# Autodesk Inventor assembly: POM_T5_03
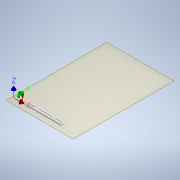
[picture p0: Inventor's stored thumbnail of the model, 180x180]
Saved by Autodesk Inventor 2020 (Build 240168000, 168)
## iProperties
Created: 2021-08-27
Part Number: POM_T5_03
Document SubType Name: Assembly
Designer: Masato
Author: Masato
## Documents named in this file (6)
- C:\Inventor\OpenPlatform_ver3_0\cam\POM_T5_03.iam
- C:\Inventor\OpenPlatform_ver3_0\cam\Disposable_Board.ipt
- C:\Inventor\OpenPlatform_ver3_0\JIG\BackLink_diagonal_jig.ipt
- C:\Inventor\OpenPlatform_ver3_0\JIG\FrontLink_diagonal_jig.ipt
- C:\Inventor\OpenPlatform_ver3_0\JIG\Foot_root_block_JIG.ipt
- C:\Inventor\OpenPlatform_ver3_0\JIG\Leg_joint_yaw_frame_JIG.ipt
## Components (5 placed, 5 different names)
1. Disposable_Board:1 — メイト:2, メイト:1, フラッシュ:1, フラッシュ:2, メイト:7, フラッシュ:6, メイト:17, フラッシュ:7, メイト:22, フラッシュ:8, メイト:27, フラッシュ:9, フラッシュ:10
2. FrontLink_diagonal_jig:1 — メイト:7, フラッシュ:6, メイト:18, メイト:28
3. BackLink_diagonal_jig:2 — メイト:17, フラッシュ:7, メイト:18
4. Foot_root_block_JIG:1 — メイト:22, フラッシュ:8, メイト:28, メイト:29
5. Leg_joint_yaw_frame_JIG:1 — メイト:27, フラッシュ:9, フラッシュ:10, メイト:29
## Relationships (16: Mate 9, Flush 7)
- メイト:2 [Mate]: Disposable_Board:1
- メイト:1 [Mate]: Disposable_Board:1
- フラッシュ:1 [Flush]: Disposable_Board:1
- フラッシュ:2 [Flush]: Disposable_Board:1
- メイト:7 [Mate]: Disposable_Board:1 ↔ FrontLink_diagonal_jig:1
- フラッシュ:6 [Flush] (2.5 mm): Disposable_Board:1 ↔ FrontLink_diagonal_jig:1
- メイト:17 [Mate]: Disposable_Board:1 ↔ BackLink_diagonal_jig:2
- フラッシュ:7 [Flush] (2.5 mm): Disposable_Board:1 ↔ BackLink_diagonal_jig:2
- メイト:18 [Mate] (2.5 mm): FrontLink_diagonal_jig:1 ↔ BackLink_diagonal_jig:2
- メイト:22 [Mate]: Disposable_Board:1 ↔ Foot_root_block_JIG:1
- フラッシュ:8 [Flush] (2.5 mm): Disposable_Board:1 ↔ Foot_root_block_JIG:1
- メイト:27 [Mate]: Disposable_Board:1 ↔ Leg_joint_yaw_frame_JIG:1
- フラッシュ:9 [Flush] (2.5 mm): Disposable_Board:1 ↔ Leg_joint_yaw_frame_JIG:1
- フラッシュ:10 [Flush] (2.5 mm): Disposable_Board:1 ↔ Leg_joint_yaw_frame_JIG:1
- メイト:28 [Mate] (2.5 mm): FrontLink_diagonal_jig:1 ↔ Foot_root_block_JIG:1
- メイト:29 [Mate] (2.5 mm): Foot_root_block_JIG:1 ↔ Leg_joint_yaw_frame_JIG:1
